# Autodesk Inventor assembly: belt_test]
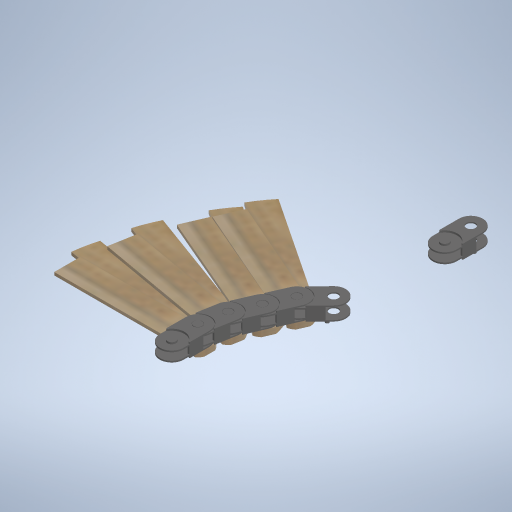
[picture p0: Inventor's stored thumbnail of the model, 512x512]
Saved by Autodesk Inventor 2024.1 (Build 281209000, 209)
## iProperties
Created: 2025-09-27
Part Number: belt_test]
Document SubType Name: Assembly
Designer: hibik
Author: hibik
## Documents named in this file (3)
- C:\Users\hibik\Documents\Robomech\conveyer\belt\belt_test].iam
- C:\Users\hibik\Documents\Robomech\conveyer\belt\belt.ipt
- C:\Users\hibik\Documents\Robomech\conveyer\belt\dish.iam
## Components (10 placed, 2 different names)
1. belt:1 — 挿入:1, 挿入:5, 角度:1
2. belt:2 — 挿入:1, 挿入:2, 挿入:6, 角度:4
3. belt:3 — 挿入:2, 挿入:3, 挿入:7, 角度:3
4. belt:4 — 挿入:3, 挿入:4, 挿入:8, 角度:2
5. belt:5 — 挿入:4
6. belt:6
7. dish:1 [sub-assembly] — 挿入:5, 角度:1
8. dish:2 [sub-assembly] — 挿入:6, 角度:4
9. dish:3 [sub-assembly] — 挿入:7, 角度:3
10. dish:4 [sub-assembly] — 挿入:8, 角度:2
## Relationships (12: Insert 8, Angle 4)
- 挿入:1 [Insert] (0.6 mm): belt:1 ↔ belt:2
- 挿入:2 [Insert] (0.6 mm): belt:2 ↔ belt:3
- 挿入:3 [Insert] (0.6 mm): belt:3 ↔ belt:4
- 挿入:4 [Insert] (0.6 mm): belt:4 ↔ belt:5
- 挿入:5 [Insert]: belt:1 ↔ dish:1
- 角度:1 [Angle] (0 deg): belt:1 ↔ dish:1
- 挿入:6 [Insert]: belt:2 ↔ dish:2
- 挿入:7 [Insert]: belt:3 ↔ dish:3
- 挿入:8 [Insert]: belt:4 ↔ dish:4
- 角度:2 [Angle] (0 deg): belt:4 ↔ dish:4
- 角度:3 [Angle] (0 deg): belt:3 ↔ dish:3
- 角度:4 [Angle] (0 deg): belt:2 ↔ dish:2
